# Autodesk Inventor assembly: Chuck - V2
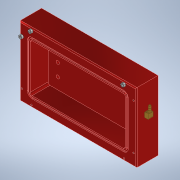
[picture p0: Inventor's stored thumbnail of the model, 180x180]
Saved by Autodesk Inventor 2022 (Build 260153000, 153)
## iProperties
Created: 2021-03-04
Part Number: Chuck - V2
Document SubType Name: Assembly
Designer: caleb
Author: caleb
## Documents named in this file (4)
- C:\Users\Caleb\Desktop\nebraska-silicon-lab\Hardware\ETL\Module Assembly\Chuck - V2\Chuck - V2.iam
- C:\Users\Caleb\Desktop\nebraska-silicon-lab\Hardware\ETL\Module Assembly\Chuck - V2\Chuck - V2.ipt
- C:\Users\Caleb\Desktop\nebraska-silicon-lab\Hardware\ETL\Module Assembly\Chuck - V2\90128A212_ZNC-PLTD ALLOY STL SCKT HEAD CAP SCREW.ipt
- C:\Users\Caleb\Desktop\nebraska-silicon-lab\Hardware\ETL\Module Assembly\Chuck - V2\44555K147_BRASS BARBED TUBE FITTING FOR VACUUM.ipt
## Components (5 placed, 3 different names)
1. Chuck - V2:1 — Insert:1, Insert:2, Insert:3, Insert:4
2. 90128A212_ZNC-PLTD ALLOY STL SCKT HEAD CAP SCREW:1 — Insert:1
3. 90128A212_ZNC-PLTD ALLOY STL SCKT HEAD CAP SCREW:2 — Insert:2
4. 90128A212_ZNC-PLTD ALLOY STL SCKT HEAD CAP SCREW:3 — Insert:3
5. 44555K147_BRASS BARBED TUBE FITTING FOR VACUUM:1 — Insert:4
## Relationships (4: Insert 4)
- Insert:1: Chuck - V2:1 ↔ 90128A212_ZNC-PLTD ALLOY STL SCKT HEAD CAP SCREW:1
- Insert:2: Chuck - V2:1 ↔ 90128A212_ZNC-PLTD ALLOY STL SCKT HEAD CAP SCREW:2
- Insert:3: Chuck - V2:1 ↔ 90128A212_ZNC-PLTD ALLOY STL SCKT HEAD CAP SCREW:3
- Insert:4: Chuck - V2:1 ↔ 44555K147_BRASS BARBED TUBE FITTING FOR VACUUM:1
